# Autodesk Inventor assembly: Base
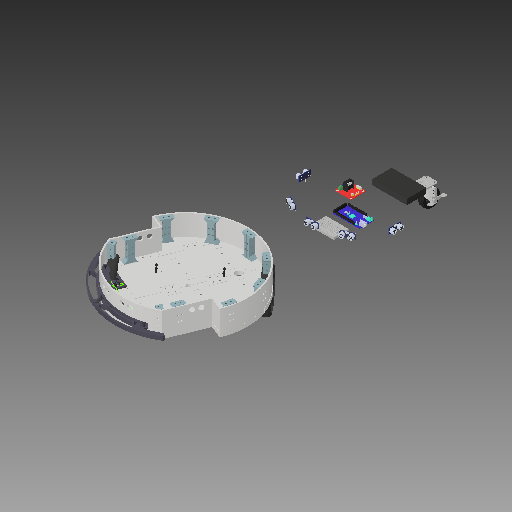
[picture p0: Inventor's stored thumbnail of the model, 512x512]
Saved by Autodesk Inventor 2017 SP1 (Build 210196100, 196)
## iProperties
Created: 2017-03-11
Part Number: Base
Document SubType Name: Assembly
Designer: zallen
Author: zallen
## Documents named in this file (18)
- C:\Users\Zach\Documents\GitHub\cr-laundry-robot\src\Base\Base.iam
- C:\Users\Zach\Documents\GitHub\cr-laundry-robot\src\Base\Swivel Wheel.ipt
- C:\Users\Zach\Documents\GitHub\cr-laundry-robot\lib\HC-SR04 Ultasonic Sensor\Sensor Ultrasónico.ipt
- C:\Users\Zach\Documents\GitHub\cr-laundry-robot\lib\Breadboard\breadboard_350_pos_asm.iam
- C:\Users\Zach\Documents\GitHub\cr-laundry-robot\lib\Arduino Mega 2560\Arduino Mega 2560.ipt
- C:\Users\Zach\Documents\GitHub\cr-laundry-robot\lib\L298n\Драйвер двигателей L298N.ipt
- C:\Users\Zach\Documents\GitHub\cr-laundry-robot\src\Base\Drive Wheel Assembly\DriveAssembly.iam
- C:\Users\Zach\Documents\GitHub\cr-laundry-robot\src\Base\Design Accelerator\Bolted Connection2.iam
- C:\Users\Zach\Documents\GitHub\cr-laundry-robot\src\Base\Design Accelerator\Bolted Connection3.iam
- C:\Users\Zach\Documents\GitHub\cr-laundry-robot\src\Base\Design Accelerator\Bolted Connection4.iam
- C:\Users\Zach\Documents\GitHub\cr-laundry-robot\src\Base\Design Accelerator\Bolted Connection5.iam
- C:\Users\Zach\Documents\GitHub\cr-laundry-robot\src\Base\Battery Pack Assembly\BatteryPackAssembly.iam
- C:\Users\Zach\Documents\GitHub\cr-laundry-robot\src\Base\Bumper Assembly\Bumper Assembly.iam
- C:\Users\Zach\Documents\GitHub\cr-laundry-robot\src\Base\Base\Design Accelerator\Bolted Connection1.iam
- C:\Users\Zach\Documents\GitHub\cr-laundry-robot\src\Base\Base\Design Accelerator\Bolted Connection2.iam
- C:\Users\Zach\Documents\GitHub\cr-laundry-robot\src\Base\Base\Design Accelerator\Bolted Connection3.iam
- C:\Users\Zach\Documents\GitHub\cr-laundry-robot\src\Base\Base\Design Accelerator\Bolted Connection4.iam
- C:\Users\Zach\Documents\GitHub\cr-laundry-robot\src\Base\Chassis - Modular\Chassis.iam
## Components (21 placed, 10 different names)
1. Swivel Wheel:1
2. Sensor Ultrasónico:1
3. Sensor Ultrasónico:2
4. Sensor Ultrasónico:3
5. breadboard_350_pos_asm:1 [sub-assembly]
6. Arduino Mega 2560:1
7. L298N:1
8. Sensor Ultrasónico:4
9. Sensor Ultrasónico:5
10. DriveAssembly:1 [sub-assembly] — Mate:47, Mate:48, Mate:49, Mate:50, Mate:51, Mate:52, Mate:53, Mate:54, Mate:72
11. Bolted Connection:1 [sub-assembly] — Mate:47, Mate:48, Mate:71
12. Bolted Connection:2 [sub-assembly] — Mate:49, Mate:50
13. Bolted Connection:3 [sub-assembly] — Mate:51, Mate:52
14. Bolted Connection:4 [sub-assembly] — Mate:53, Mate:54
15. BatteryPackAssembly:1 [sub-assembly]
16. Bumper Assembly:1 [sub-assembly] — Mate:58, Mate:59, Mate:60, Mate:61, Mate:62, Mate:63, Mate:64, Mate:65, Mate:67
17. Bolted Connection:5 [sub-assembly] — Mate:58, Mate:59
18. Bolted Connection:6 [sub-assembly] — Mate:60, Mate:61, Mate:70
19. Bolted Connection:7 [sub-assembly] — Mate:62, Mate:63, Mate:69
20. Bolted Connection:8 [sub-assembly] — Mate:64, Mate:65, Mate:68
21. Chassis:1 [sub-assembly] — Mate:66, Mate:67, Mate:68, Mate:69, Mate:70, Mate:71, Mate:72
## Relationships (23: Mate 23)
- Mate:47: DriveAssembly:1 ↔ Bolted Connection:1
- Mate:48: DriveAssembly:1 ↔ Bolted Connection:1
- Mate:49: DriveAssembly:1 ↔ Bolted Connection:2
- Mate:50: DriveAssembly:1 ↔ Bolted Connection:2
- Mate:51: DriveAssembly:1 ↔ Bolted Connection:3
- Mate:52: DriveAssembly:1 ↔ Bolted Connection:3
- Mate:53: DriveAssembly:1 ↔ Bolted Connection:4
- Mate:54: DriveAssembly:1 ↔ Bolted Connection:4
- Mate:58: Bumper Assembly:1 ↔ Bolted Connection:5
- Mate:59: Bumper Assembly:1 ↔ Bolted Connection:5
- Mate:60: Bumper Assembly:1 ↔ Bolted Connection:6
- Mate:61: Bumper Assembly:1 ↔ Bolted Connection:6
- Mate:62: Bumper Assembly:1 ↔ Bolted Connection:7
- Mate:63: Bumper Assembly:1 ↔ Bolted Connection:7
- Mate:64: Bumper Assembly:1 ↔ Bolted Connection:8
- Mate:65: Bumper Assembly:1 ↔ Bolted Connection:8
- Mate:66: Chassis:1
- Mate:67: Bumper Assembly:1 ↔ Chassis:1
- Mate:68: Bolted Connection:8 ↔ Chassis:1
- Mate:69: Bolted Connection:7 ↔ Chassis:1
- Mate:70: Bolted Connection:6 ↔ Chassis:1
- Mate:71: Bolted Connection:1 ↔ Chassis:1
- Mate:72: DriveAssembly:1 ↔ Chassis:1
